# Autodesk Inventor assembly: Structure
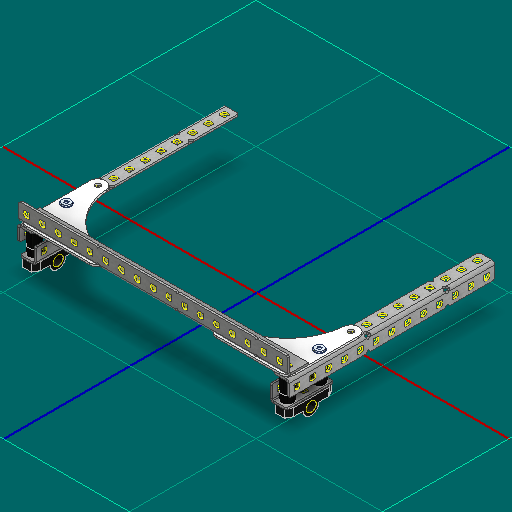
[picture p0: Inventor's stored thumbnail of the model, 512x512]
Saved by Autodesk Inventor 2025 (Build 290162000, 162)
## iProperties
Created: 2024-10-21
Part Number: Structure
Document SubType Name: Assembly
Designer: averey
Author: averey
## Documents named in this file (5)
- C:\Users\avere\VEX\High Stakes\CAD\V2\Intake\Arm\Structure.iam
- C:\Users\avere\VEX\High Stakes\CAD\V2\Intake\Arm\Left Angle Structure.iam
- C:\Users\avere\VEX\High Stakes\CAD\V2\Intake\Arm\Right Angle Structure\Right Angle Structure.iam
- C:\Users\avere\VEX\High Stakes\CAD\ROBOPROS-CAD-Inventor\Structure\C Channel\Aluminum 1x3x1 Half Thick Cut\Alu C Half Thick 1x3x1x17.ipt
- C:\Users\avere\VEX\High Stakes\CAD\V2\Intake\Arm\Custom Parts\Arm Triangle Gusset.ipt
## Components (5 placed, 4 different names)
1. Left Angle Structure:1 [sub-assembly] — Mate:1, Mate:2, Flush:1, Mate:4
2. Right Angle Structure:1 [sub-assembly] — Flush:2, Mate:3, Flush:3, Insert:1
3. Alu C Half Thick 1x3x1x17:1 — Insert:1, Mate:4, Insert:2, Mate:5, Insert:3, Mate:6
4. Arm Triangle Gusset:1 — Insert:2, Mate:5
5. Arm Triangle Gusset:2 — Insert:3, Mate:6
## Relationships (12: Mate 6, Flush 3, Insert 3)
- Mate:1 (96.4184 mm): Left Angle Structure:1
- Mate:2 (-82.55 mm): Left Angle Structure:1
- Flush:1: Left Angle Structure:1
- Flush:2: Right Angle Structure:1
- Mate:3 (-82.55 mm): Right Angle Structure:1
- Flush:3 (96.4184 mm): Right Angle Structure:1
- Insert:1 (1.5875 mm): Right Angle Structure:1 ↔ Alu C Half Thick 1x3x1x17:1
- Mate:4: Left Angle Structure:1 ↔ Alu C Half Thick 1x3x1x17:1
- Insert:2: Alu C Half Thick 1x3x1x17:1 ↔ Arm Triangle Gusset:1
- Mate:5: Alu C Half Thick 1x3x1x17:1 ↔ Arm Triangle Gusset:1
- Insert:3: Alu C Half Thick 1x3x1x17:1 ↔ Arm Triangle Gusset:2
- Mate:6: Alu C Half Thick 1x3x1x17:1 ↔ Arm Triangle Gusset:2
